# Autodesk Inventor assembly: eESTRUTURA
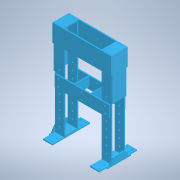
[picture p0: Inventor's stored thumbnail of the model, 180x180]
Saved by Autodesk Inventor 2021 (Build 250183000, 183)
## iProperties
Created: 2020-01-15
Part Number: eESTRUTURA
Document SubType Name: Assembly
Designer: Nelson
Sending System: SolidWorks 2020
Last Author: Micro
Last Saved: 2020-01-15
Author: Nelson
## Documents named in this file (10)
- D:\Nelson\Documentos\Inventor\PrensaHidraulica_Automatizada\Estructura.iam
- D:\Nelson\Documentos\Inventor\PrensaHidraulica_Automatizada\PH 001.ipt
- D:\Nelson\Documentos\Inventor\PrensaHidraulica_Automatizada\PH 003.ipt
- D:\Nelson\Documentos\Inventor\PrensaHidraulica_Automatizada\PH 004.ipt
- D:\Nelson\Documentos\Inventor\PrensaHidraulica_Automatizada\PH 009.ipt
- D:\Nelson\Documentos\Inventor\PrensaHidraulica_Automatizada\PH 008.ipt
- D:\Nelson\Documentos\Inventor\PrensaHidraulica_Automatizada\PH 005.ipt
- D:\Nelson\Documentos\Inventor\PrensaHidraulica_Automatizada\PH 007.ipt
- D:\Nelson\Documentos\Inventor\PrensaHidraulica_Automatizada\PH 011.ipt
- D:\Nelson\Documentos\Inventor\PrensaHidraulica_Automatizada\PH 012.ipt
## Components (21 placed, 9 different names)
1. PH 001:1 — Mate:3, Mate:4, Flush:5, Flush:21, Mate:19, Flush:22, Mate:24, Flush:28, Mate:31
2. PH 003:1 — Mate:2, Flush:3, Flush:4, Mate:4, Flush:5, Mate:6
3. PH 003:2 — Mate:18, Mate:24, Flush:28
4. PH 001:2 — Mate:5, Mate:6, Flush:6, Mate:21, Mate:25, Flush:29, Mate:27
5. PH 004:1 — Mate:18, Flush:21, Mate:19, Flush:22, Flush:26
6. PH 009:1 — Mate:2, Flush:3, Flush:4, Mate:3, Mate:5, Flush:6, Mate:7, Flush:7, Flush:8, Mate:10, Flush:10, Flush:11
7. PH 008:1 — Mate:7, Flush:7, Flush:8
8. PH 005:1 — Mate:21, Flush:25, Flush:26
9. PH 005:2 — Mate:20, Flush:24, Flush:30, Flush:33
10. PH 007:1 — Mate:25, Flush:29, Flush:30
11. PH 001:3 — Mate:14, Mate:15, Flush:15, Mate:17, Flush:20, Mate:20, Flush:27, Mate:29, Mate:30, Flush:33
12. PH 003:4 — Mate:11, Flush:12, Flush:13, Mate:13, Flush:14, Mate:15
13. PH 003:5 — Mate:22, Mate:23, Flush:27
14. PH 001:4 — Mate:12, Mate:13, Flush:14, Mate:22, Mate:26, Mate:28, Flush:25, Flush:19
15. PH 004:2 — Mate:17, Flush:19, Flush:20, Flush:24, Mate:23
16. PH 009:2 — Mate:10, Flush:10, Flush:11, Mate:11, Flush:12, Flush:13, Mate:12, Mate:14, Flush:15, Mate:16, Flush:16, Flush:17
17. PH 008:2 — Mate:16, Flush:16, Flush:17
18. PH 011:1 — Mate:26, Mate:27, Mate:28, Mate:32, Flush:31, Mate:33, Flush:32
19. PH 011:2 — Mate:29, Mate:30, Mate:31, Mate:34, Mate:35
20. PH 012:1 — Mate:32, Flush:31, Mate:34
21. PH 012:2 — Mate:33, Flush:32, Mate:35
## Relationships (60: Mate 32, Flush 28)
- Mate:2: PH 003:1 ↔ PH 009:1
- Flush:3: PH 003:1 ↔ PH 009:1
- Flush:4 (275 mm): PH 003:1 ↔ PH 009:1
- Mate:3: PH 001:1 ↔ PH 009:1
- Mate:4: PH 001:1 ↔ PH 003:1
- Flush:5: PH 001:1 ↔ PH 003:1
- Mate:5: PH 001:2 ↔ PH 009:1
- Mate:6: PH 003:1 ↔ PH 001:2
- Flush:6: PH 001:2 ↔ PH 009:1
- Mate:7: PH 009:1 ↔ PH 008:1
- Flush:7: PH 009:1 ↔ PH 008:1
- Flush:8 (150 mm): PH 009:1 ↔ PH 008:1
- Mate:10 (800 mm): PH 009:1 ↔ PH 009:2
- Flush:10: PH 009:1 ↔ PH 009:2
- Flush:11: PH 009:1 ↔ PH 009:2
- Mate:11: PH 003:4 ↔ PH 009:2
- Flush:12: PH 003:4 ↔ PH 009:2
- Flush:13 (275 mm): PH 003:4 ↔ PH 009:2
- Mate:12: PH 001:4 ↔ PH 009:2
- Mate:13: PH 003:4 ↔ PH 001:4
- Flush:14: PH 003:4 ↔ PH 001:4
- Mate:14: PH 001:3 ↔ PH 009:2
- Mate:15: PH 001:3 ↔ PH 003:4
- Flush:15: PH 001:3 ↔ PH 009:2
- Mate:16: PH 009:2 ↔ PH 008:2
- Flush:16: PH 009:2 ↔ PH 008:2
- Flush:17 (150 mm): PH 009:2 ↔ PH 008:2
- Mate:17: PH 001:3 ↔ PH 004:2
- Flush:19: PH 001:4 ↔ PH 004:2
- Flush:20: PH 001:3 ↔ PH 004:2
- Mate:18: PH 003:2 ↔ PH 004:1
- Flush:21: PH 001:1 ↔ PH 004:1
- Mate:19: PH 001:1 ↔ PH 004:1
- Flush:22: PH 001:1 ↔ PH 004:1
- Mate:20: PH 005:2 ↔ PH 001:3
- Flush:24: PH 005:2 ↔ PH 004:2
- Mate:21: PH 001:2 ↔ PH 005:1
- Flush:25: PH 005:1 ↔ PH 001:4
- Flush:26: PH 004:1 ↔ PH 005:1
- Mate:22: PH 003:5 ↔ PH 001:4
- Mate:23: PH 003:5 ↔ PH 004:2
- Flush:27: PH 001:3 ↔ PH 003:5
- Mate:24: PH 001:1 ↔ PH 003:2
- Flush:28: PH 001:1 ↔ PH 003:2
- Mate:25: PH 001:2 ↔ PH 007:1
- Flush:29: PH 001:2 ↔ PH 007:1
- Flush:30: PH 005:2 ↔ PH 007:1
- Mate:26: PH 001:4 ↔ PH 011:1
- Mate:27: PH 001:2 ↔ PH 011:1
- Mate:28: PH 001:4 ↔ PH 011:1
- Mate:29: PH 001:3 ↔ PH 011:2
- Mate:30: PH 001:3 ↔ PH 011:2
- Mate:31: PH 001:1 ↔ PH 011:2
- Mate:32: PH 011:1 ↔ PH 012:1
- Flush:31: PH 011:1 ↔ PH 012:1
- Mate:33: PH 011:1 ↔ PH 012:2
- Flush:32: PH 011:1 ↔ PH 012:2
- Mate:34 (162.3 mm): PH 011:2 ↔ PH 012:1
- Mate:35 (162.3 mm): PH 011:2 ↔ PH 012:2
- Flush:33: PH 005:2 ↔ PH 001:3
